# Autodesk Inventor assembly: GreyT Telescope Bottom Block
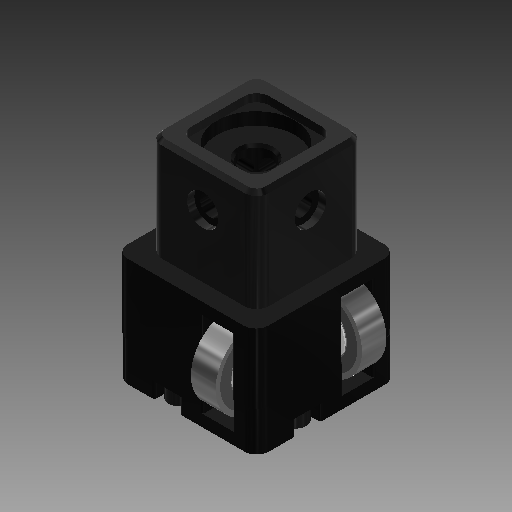
[picture p0: Inventor's stored thumbnail of the model, 512x512]
Saved by Autodesk Inventor 2023 (Build 270158000, 158)
## iProperties
Created: 2021-12-31
Part Number: GreyT Telescope Bottom Block
Document SubType Name: Assembly
Mass: 81.1813 g
Surface Area: 189.917 cm^2
Volume: 22.0375 cm^3
Density: 3.68377 g/cm^3
Revision Number: ANY
## Documents named in this file (11)
- E:\Collaborative Robots\Collaborative Part Library\Elevators\GreyT Telescope\1 in Bottom Block WCP-0418.iam
- E:\Collaborative Robots\Collaborative Part Library\Elevators\GreyT Telescope\Smallest Stage\WCP-0418-006 Rev1.ipt
- E:\Collaborative Robots\Collaborative Part Library\Elevators\GreyT Telescope\Smallest Stage\WCP-0418-007 Rev1.ipt
- E:\Collaborative Robots\Collaborative Part Library\Elevators\GreyT Telescope\WCP-0039 Rev1.ipt
- E:\Collaborative Robots\Collaborative Part Library\Elevators\GreyT Telescope\Smallest Stage\WCP-0383 Rev1.ipt
- E:\Collaborative Robots\Collaborative Part Library\Hardware\Fasteners\Machine Screws\4-40 UNCx0.5 Socket Head Cap Screw.ipt
- C:\Users\Cal\Desktop\Robotics\Design\Collaborative\Collaborative Parts Library\Hardware\Fasteners\Machine Screws.ipt
- E:\Collaborative Robots\Collaborative Part Library\Power Transfer\Bearings and Bushings\Bearings\R4.ipt
- C:\Users\Cal\Desktop\Robotics\Design\Collaborative\Collaborative Parts Library\Power Transfer\Bearings and Bushings\Bearings.ipt
- E:\Collaborative Robots\Collaborative Part Library\Hardware\Dowel Pins\Dowel Pins\0.25in  x 0.375in Stainless Steel Dowel Pin.ipt
- C:\Users\Cal\Desktop\Robotics\Design\Collaborative\Collaborative Parts Library\Hardware\Dowel Pins\Dowel Pins.ipt
## Components (23 placed, 7 different names)
1. WCP-0418-006 Rev1:1 — Insert:1, Angle:1, Tangent:1, Mate:2, Tangent:2, Insert:8, Angle:2, Flush:1, Flush:2
2. WCP-0418-007 Rev1_1068 — Insert:2, Insert:3, Insert:4, Insert:5, Insert:8, Angle:2, Mate:3
3. 4-40 UNCx0.5 Socket Head Cap Screw:1 — Insert:3
4. 4-40 UNCx0.5 Socket Head Cap Screw:2 — Insert:4
5. 4-40 UNCx0.5 Socket Head Cap Screw:3 — Insert:5
6. 4-40 UNCx0.5 Socket Head Cap Screw:4 — Insert:2
7. WCP-0383 Rev1_1089 — Insert:1, Angle:1
8. 0.25in  x 0.375in Stainless Steel Dowel Pin:1 — Mate:1, Tangent:1, Mate:2, Tangent:2
9. WCP-0039 Rev1:8 — Insert:7, Symmetry:1
10. R4:1 — Insert:6, Insert:7, Mate:1
11. WCP-0039 Rev1:7 — Insert:6, Symmetry:1
12. 0.25in  x 0.375in Stainless Steel Dowel Pin:2
13. WCP-0039 Rev1:9
14. R4:2
15. WCP-0039 Rev1:10
16. 0.25in  x 0.375in Stainless Steel Dowel Pin:3
17. WCP-0039 Rev1:11
18. R4:3
19. WCP-0039 Rev1:12
20. 0.25in  x 0.375in Stainless Steel Dowel Pin:4
21. WCP-0039 Rev1:13
22. R4:4
23. WCP-0039 Rev1:14
## Component patterns: (4 elements, first: 0.25in  x 0.375in Stainless Steel Dowel Pin:1 + WCP-0039 Rev1:8 + R4:1 + WCP-0039 Rev1:7)
## Relationships (18: Insert 8, Mate 3, Angle 2, Tangent 2, Flush 2, Symmetry 1)
- Insert:1: WCP-0418-006 Rev1:1 ↔ WCP-0383 Rev1_1089
- Angle:1 (0 deg): WCP-0418-006 Rev1:1 ↔ WCP-0383 Rev1_1089
- Insert:2: WCP-0418-007 Rev1_1068 ↔ 4-40 UNCx0.5 Socket Head Cap Screw:4
- Insert:3: WCP-0418-007 Rev1_1068 ↔ 4-40 UNCx0.5 Socket Head Cap Screw:1
- Insert:4: WCP-0418-007 Rev1_1068 ↔ 4-40 UNCx0.5 Socket Head Cap Screw:2
- Insert:5: WCP-0418-007 Rev1_1068 ↔ 4-40 UNCx0.5 Socket Head Cap Screw:3
- Insert:6: R4:1 ↔ WCP-0039 Rev1:7
- Insert:7: WCP-0039 Rev1:8 ↔ R4:1
- Mate:1: 0.25in  x 0.375in Stainless Steel Dowel Pin:1 ↔ R4:1
- Symmetry:1: WCP-0039 Rev1:8 ↔ WCP-0039 Rev1:7
- Tangent:1: WCP-0418-006 Rev1:1 ↔ 0.25in  x 0.375in Stainless Steel Dowel Pin:1
- Mate:2: WCP-0418-006 Rev1:1 ↔ 0.25in  x 0.375in Stainless Steel Dowel Pin:1
- Tangent:2: WCP-0418-006 Rev1:1 ↔ 0.25in  x 0.375in Stainless Steel Dowel Pin:1
- Insert:8: WCP-0418-006 Rev1:1 ↔ WCP-0418-007 Rev1_1068
- Angle:2 (0 deg): WCP-0418-006 Rev1:1 ↔ WCP-0418-007 Rev1_1068
- Mate:3: WCP-0418-007 Rev1_1068
- Flush:1: WCP-0418-006 Rev1:1
- Flush:2: WCP-0418-006 Rev1:1
